# Autodesk Inventor assembly: цепь_MIR4_MIR
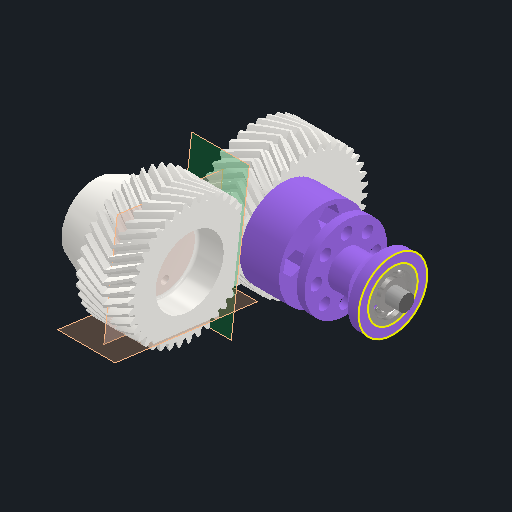
[picture p0: Inventor's stored thumbnail of the model, 512x512]
Saved by Autodesk Inventor 2026.2 (Build 302298000, 298)
## iProperties
Created: 2024-07-09
Part Number: цепь_MIR4_MIR
Document SubType Name: Assembly
Designer: Phantom
Author: Phantom
## Documents named in this file (6)
- C:\Users\Phantom\Desktop\Phantom16950\цепь_MIR4_MIR.iam
- C:\Users\Phantom\Desktop\Phantom16950\втулка для подш 2 часть_MIR6_MIR.ipt
- C:\Users\Phantom\Desktop\Phantom16950\втулка для подш_MIR6_MIR.ipt
- C:\Users\Phantom\Desktop\Phantom16950\Деталь_64_MIR6_MIR.ipt
- C:\Users\Phantom\Desktop\Phantom16950\BS 290 SKF - SKF 626-RZ_MIR6_MIR.ipt
- C:\Users\Phantom\Desktop\Phantom16950\цепь\Мастер проектирования\Цилиндрическое зубчатое зацепление4_MIR_MIR.iam
## Components (6 placed, 5 different names)
1. втулка для подш 2 часть_MIR6_MIR:1 — Совмещение:16, Совмещение:23, Совмещение:20
2. втулка для подш_MIR6_MIR:1 — Совмещение:16, Совмещение:17, Совмещение:25
3. Деталь_64_MIR6_MIR:1 — Совмещение:17, Совмещение:23, Совмещение:21, Совмещение:19
4. BS 290 SKF - SKF 626-RZ_MIR6_MIR:1 — Совмещение:20, Совмещение:21
5. BS 290 SKF - SKF 626-RZ_MIR6_MIR:2 — Совмещение:19, Совмещение:27
6. Цилиндрическое зубчатое зацепление4_MIR_MIR:1 [sub-assembly] — Совмещение:25, Совмещение:27
## Relationships (8: Mate 8)
- Совмещение:16 [Mate]: втулка для подш 2 часть_MIR6_MIR:1 ↔ втулка для подш_MIR6_MIR:1
- Совмещение:17 [Mate]: втулка для подш_MIR6_MIR:1 ↔ Деталь_64_MIR6_MIR:1
- Совмещение:23 [Mate]: втулка для подш 2 часть_MIR6_MIR:1 ↔ Деталь_64_MIR6_MIR:1
- Совмещение:20 [Mate]: втулка для подш 2 часть_MIR6_MIR:1 ↔ BS 290 SKF - SKF 626-RZ_MIR6_MIR:1
- Совмещение:21 [Mate]: Деталь_64_MIR6_MIR:1 ↔ BS 290 SKF - SKF 626-RZ_MIR6_MIR:1
- Совмещение:19 [Mate]: Деталь_64_MIR6_MIR:1 ↔ BS 290 SKF - SKF 626-RZ_MIR6_MIR:2
- Совмещение:25 [Mate]: втулка для подш_MIR6_MIR:1 ↔ Цилиндрическое зубчатое зацепление4_MIR_MIR:1
- Совмещение:27 [Mate]: BS 290 SKF - SKF 626-RZ_MIR6_MIR:2 ↔ Цилиндрическое зубчатое зацепление4_MIR_MIR:1
